# Autodesk Inventor assembly: reducer_2
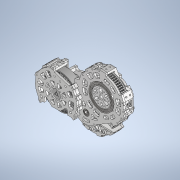
[picture p0: Inventor's stored thumbnail of the model, 180x180]
Saved by Autodesk Inventor 2020 (Build 240168000, 168)
## iProperties
Created: 2020-07-04
Part Number: reducer_2
Document SubType Name: Assembly
Designer: psrobotics
Author: psrobotics
## Documents named in this file (20)
- D:\projects-3\biped_gen1\hardware\reducer_2.iam
- D:\projects-3\biped_gen1\hardware\90_motor.iam
- D:\projects-3\biped_gen1\hardware\xl_20.ipt
- D:\projects-3\biped_gen1\hardware\xl_wheel_ass.iam
- D:\projects-3\biped_gen1\hardware\xl_60_out_2.ipt
- D:\projects-3\biped_gen1\hardware\bearing_6810zz.ipt
- D:\projects-3\biped_gen1\hardware\shell_2.ipt
- D:\projects-3\biped_gen1\hardware\shell_3.ipt
- D:\projects-3\biped_gen1\hardware\shell_4.ipt
- D:\projects-3\biped_gen1\hardware\motor_h_1.ipt
- D:\projects-3\biped_gen1\hardware\motor_h_2.ipt
- D:\projects-3\biped_gen1\hardware\shell_5.ipt
- D:\projects-3\biped_gen1\hardware\motor_h_3.ipt
- D:\projects-3\biped_gen1\hardware\bearing_shell_1.ipt
- D:\projects-3\biped_gen1\hardware\bearing_shell_2.ipt
- D:\projects-3\biped_gen1\hardware\bearing_8_16_5.ipt
- D:\projects-3\biped_gen1\hardware\bearing_6_13_5.ipt
- D:\projects-3\biped_gen1\hardware\encoder_ma_holder_1.ipt
- D:\projects-3\biped_gen1\hardware\encoder_ma.ipt
- D:\projects-3\biped_gen1\hardware\motor_pin_shell_1.ipt
## Components (23 placed, 19 different names)
1. 90_motor:1 [sub-assembly] — Insert:1, Insert:2, Tangent:3, Flush:4, Insert:29, Insert:38
2. xl_20:1 — Insert:1, Insert:2, Flush:1, Tangent:1
3. xl_wheel_ass:1 [sub-assembly] — Flush:1, Tangent:1, Flush:2, Tangent:2, Insert:9
4. xl_60_out_2:1 — Flush:2, Tangent:2, Tangent:3, Insert:4, Insert:7, Insert:8
5. bearing_6810zz:1 — Insert:4
6. shell_2:1 — Angle:1, Insert:9, Insert:18
7. shell_2:3 — Insert:7, Angle:1, Angle:2, Flush:7, Insert:14, Insert:17
8. shell_2:4 — Insert:8, Angle:2, Flush:6, Insert:15, Insert:16, Insert:19, Insert:20
9. shell_3:1 — Flush:4, Flush:5, Insert:23, Insert:24, Insert:25, Insert:26
10. shell_4:1 — Flush:5, Insert:25, Insert:26
11. motor_h_1:1 — Flush:6, Insert:12, Insert:13, Insert:14, Insert:15, Insert:16, Insert:17, Insert:18, Flush:10, Insert:27, Insert:28, Insert:30, Insert:31
12. motor_h_2:1 — Flush:7, Flush:8, Insert:19, Insert:20, Insert:21, Insert:22, Insert:32
13. shell_5:1 — Flush:8, Flush:9, Insert:10, Insert:11, Insert:21, Insert:22
14. motor_h_3:1 — Flush:9, Insert:10, Insert:11, Insert:23, Insert:24, Insert:29
15. bearing_shell_1:1 — Insert:12, Insert:13
16. bearing_shell_2:1 — Flush:10, Insert:27, Insert:28, Insert:40, Flush:11, Insert:42, Insert:43
17. bearing_8_16_5:1 — Insert:30
18. bearing_8_16_5:2 — Insert:32
19. bearing_8_16_5:3 — Insert:31
20. bearing_6_13_5:1 — Insert:40
21. encoder_ma_holder_1:1 — Insert:38, Insert:41
22. encoder_ma:1 — Insert:41
23. motor_pin_shell_1:1 — Flush:11, Insert:42, Insert:43
## Relationships (49: Insert 34, Flush 10, Tangent 3, Angle 2)
- Insert:1: 90_motor:1 ↔ xl_20:1
- Insert:2: 90_motor:1 ↔ xl_20:1
- Flush:1: xl_20:1 ↔ xl_wheel_ass:1
- Tangent:1 (1.3 mm): xl_20:1 ↔ xl_wheel_ass:1
- Flush:2: xl_wheel_ass:1 ↔ xl_60_out_2:1
- Tangent:2 (1.3 mm): xl_wheel_ass:1 ↔ xl_60_out_2:1
- Tangent:3 (20 mm): 90_motor:1 ↔ xl_60_out_2:1
- Insert:4: xl_60_out_2:1 ↔ bearing_6810zz:1
- Insert:7 (-0.5 mm): xl_60_out_2:1 ↔ shell_2:3
- Angle:1 (160 deg): shell_2:1 ↔ shell_2:3
- Insert:8 (-0.5 mm): xl_60_out_2:1 ↔ shell_2:4
- Angle:2 (230 deg): shell_2:3 ↔ shell_2:4
- Insert:9 (-0.5 mm): xl_wheel_ass:1 ↔ shell_2:1
- Flush:4: 90_motor:1 ↔ shell_3:1
- Flush:5: shell_3:1 ↔ shell_4:1
- Flush:6: shell_2:4 ↔ motor_h_1:1
- Flush:7: shell_2:3 ↔ motor_h_2:1
- Flush:8: motor_h_2:1 ↔ shell_5:1
- Flush:9: shell_5:1 ↔ motor_h_3:1
- Insert:10: shell_5:1 ↔ motor_h_3:1
- Insert:11: shell_5:1 ↔ motor_h_3:1
- Insert:12: motor_h_1:1 ↔ bearing_shell_1:1
- Insert:13: motor_h_1:1 ↔ bearing_shell_1:1
- Insert:14: shell_2:3 ↔ motor_h_1:1
- Insert:15: shell_2:4 ↔ motor_h_1:1
- Insert:16: shell_2:4 ↔ motor_h_1:1
- Insert:17: shell_2:3 ↔ motor_h_1:1
- Insert:18: shell_2:1 ↔ motor_h_1:1
- Insert:19: shell_2:4 ↔ motor_h_2:1
- Insert:20: shell_2:4 ↔ motor_h_2:1
- Insert:21: motor_h_2:1 ↔ shell_5:1
- Insert:22: motor_h_2:1 ↔ shell_5:1
- Insert:23: shell_3:1 ↔ motor_h_3:1
- Insert:24: shell_3:1 ↔ motor_h_3:1
- Insert:25: shell_3:1 ↔ shell_4:1
- Insert:26: shell_3:1 ↔ shell_4:1
- Flush:10: motor_h_1:1 ↔ bearing_shell_2:1
- Insert:27: motor_h_1:1 ↔ bearing_shell_2:1
- Insert:28: motor_h_1:1 ↔ bearing_shell_2:1
- Insert:29: 90_motor:1 ↔ motor_h_3:1
- Insert:30: motor_h_1:1 ↔ bearing_8_16_5:1
- Insert:31: motor_h_1:1 ↔ bearing_8_16_5:3
- Insert:32: motor_h_2:1 ↔ bearing_8_16_5:2
- Insert:38: 90_motor:1 ↔ encoder_ma_holder_1:1
- Insert:40: bearing_shell_2:1 ↔ bearing_6_13_5:1
- Insert:41: encoder_ma_holder_1:1 ↔ encoder_ma:1
- Flush:11: bearing_shell_2:1 ↔ motor_pin_shell_1:1
- Insert:42: bearing_shell_2:1 ↔ motor_pin_shell_1:1
- Insert:43: bearing_shell_2:1 ↔ motor_pin_shell_1:1
